# Autodesk Inventor assembly: NavCom
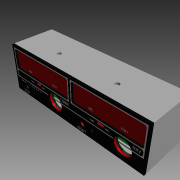
[picture p0: Inventor's stored thumbnail of the model, 180x180]
Saved by Autodesk Inventor 2014 (Build 180170000, 170)
## iProperties
Created: 2017-02-12
Part Number: NavCom
Document SubType Name: Assembly
Designer: N
Author: N
## Documents named in this file (7)
- D:\Projekty\RadioStack_v2\trunk\Draw_Inventor\NavCom.iam
- D:\Projekty\RadioStack_v2\trunk\Draw_Inventor\NavCom_mask.ipt
- D:\Projekty\RadioStack_v2\trunk\Draw_Inventor\NavCom_plexi.ipt
- D:\Projekty\RadioStack_v2\trunk\Draw_Inventor\NavCom_panel.ipt
- D:\Projekty\RadioStack_v2\trunk\Draw_Inventor\NavCom_PCB.ipt
- D:\Projekty\RadioStack_v2\trunk\Draw_Inventor\Krabicka_dolna_cast.ipt
- D:\Projekty\RadioStack_v2\trunk\Draw_Inventor\NavCom_Box_Upper_Part.ipt
## Components (8 placed, 6 different names)
1. NavCom_mask:1 — Stejný směr:1, Stejný směr:5, Proti sobě:4
2. NavCom_plexi:1 — Stejný směr:1, Stejný směr:2, Stejný směr:3, Stejný směr:4, Stejný směr:5, Stejný směr:6, Stejný směr:7, Stejný směr:8, Proti sobě:4, Stejný směr:9, Stejný směr:10, Proti sobě:10
3. NavCom_panel:1 — Stejný směr:9, Stejný směr:10, Stejný směr:11, Stejný směr:12, Proti sobě:5, Proti sobě:6, Proti sobě:10
4. NavCom_PCB:2 — Stejný směr:2, Stejný směr:6, Proti sobě:6, Proti sobě:7
5. NavCom_PCB:3 — Stejný směr:3, Stejný směr:7, Proti sobě:7, Proti sobě:8
6. NavCom_PCB:4 — Stejný směr:4, Stejný směr:8, Proti sobě:8
7. Krabicka_dolna_cast:1 — Stejný směr:11, Stejný směr:12, Proti sobě:5, Stejný směr:13, Stejný směr:14, Proti sobě:9
8. NavCom_Box_Upper_Part:1 — Stejný směr:13, Stejný směr:14, Proti sobě:9
## Relationships (21: Flush 14, Mate 7)
- Stejný směr:1 [Flush]: NavCom_mask:1 ↔ NavCom_plexi:1
- Stejný směr:2 [Flush]: NavCom_plexi:1 ↔ NavCom_PCB:2
- Stejný směr:3 [Flush]: NavCom_plexi:1 ↔ NavCom_PCB:3
- Stejný směr:4 [Flush]: NavCom_plexi:1 ↔ NavCom_PCB:4
- Stejný směr:5 [Flush]: NavCom_mask:1 ↔ NavCom_plexi:1
- Stejný směr:6 [Flush]: NavCom_plexi:1 ↔ NavCom_PCB:2
- Stejný směr:7 [Flush]: NavCom_plexi:1 ↔ NavCom_PCB:3
- Stejný směr:8 [Flush]: NavCom_plexi:1 ↔ NavCom_PCB:4
- Proti sobě:4 [Mate]: NavCom_mask:1 ↔ NavCom_plexi:1
- Stejný směr:9 [Flush]: NavCom_plexi:1 ↔ NavCom_panel:1
- Stejný směr:10 [Flush]: NavCom_plexi:1 ↔ NavCom_panel:1
- Stejný směr:11 [Flush]: NavCom_panel:1 ↔ Krabicka_dolna_cast:1
- Stejný směr:12 [Flush]: NavCom_panel:1 ↔ Krabicka_dolna_cast:1
- Proti sobě:5 [Mate]: NavCom_panel:1 ↔ Krabicka_dolna_cast:1
- Proti sobě:6 [Mate] (11.43 mm): NavCom_panel:1 ↔ NavCom_PCB:2
- Proti sobě:7 [Mate] (10.795 mm): NavCom_PCB:2 ↔ NavCom_PCB:3
- Proti sobě:8 [Mate] (10.795 mm): NavCom_PCB:3 ↔ NavCom_PCB:4
- Stejný směr:13 [Flush]: Krabicka_dolna_cast:1 ↔ NavCom_Box_Upper_Part:1
- Stejný směr:14 [Flush]: Krabicka_dolna_cast:1 ↔ NavCom_Box_Upper_Part:1
- Proti sobě:9 [Mate]: Krabicka_dolna_cast:1 ↔ NavCom_Box_Upper_Part:1
- Proti sobě:10 [Mate]: NavCom_plexi:1 ↔ NavCom_panel:1
